# Autodesk Inventor assembly: !drivebay
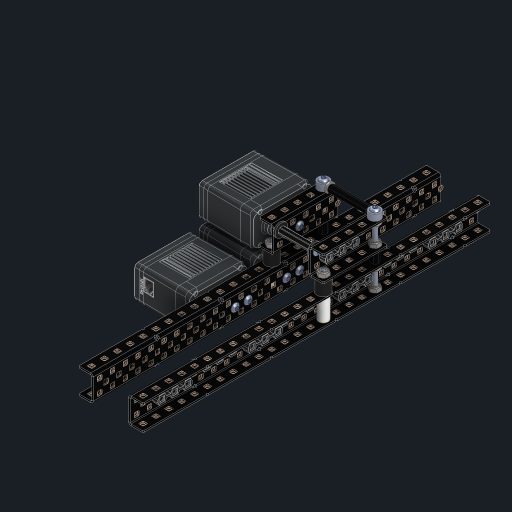
[picture p0: Inventor's stored thumbnail of the model, 512x512]
Saved by Autodesk Inventor 2024 (Build 280153000, 153)
## iProperties
Created: 2024-03-11
Part Number: !drivebay
Document SubType Name: Assembly
Designer: Averey Ku
Author: Averey Ku
## Documents named in this file (10)
- D:\vex_robotics\hardware\cad\eca\chassis\drivebay\!drivebay.iam
- D:\vex_robotics\hardware\cad\eca\chassis\drivebay\inner.iam
- D:\vex_robotics\hardware\cad\eca\chassis\drivebay\outer.iam
- D:\vex_robotics\hardware\cad\VEX-CAD-Inventor-1.41\Motion\Shaft LS\Shaft Collar ipts\Shaft Collar No Screw.ipt
- D:\vex_robotics\hardware\cad\VEX-CAD-Inventor-1.41\Structure\Standoff\Standoff 1.25.ipt
- D:\vex_robotics\hardware\cad\VEX-CAD-Inventor-1.41\Structure\Standoff\Standoff 1.50.ipt
- D:\vex_robotics\hardware\cad\VEX-CAD-Inventor-1.41\Structure\Standoff.ipt
- D:\vex_robotics\hardware\cad\VEX-CAD-Inventor-1.41\Motion\Spacers\Washer Delrin\DWasher .500 OD x .062500.ipt
- D:\vex_robotics\hardware\cad\VEX-CAD-Inventor-1.41\Motion\Spacers\Washer Steel\SWasher .375 OD x .062500.ipt
- D:\vex_robotics\hardware\cad\VEX-CAD-Inventor-1.41\Motion\Spacers\Washer Steel.ipt
## Components (9 placed, 7 different names)
1. inner:1 [sub-assembly] — Insert:1, Mate:1, Insert:2, Insert:8
2. outer:1 [sub-assembly] — Insert:1, Mate:1, Insert:3
3. Shaft Collar No Screw:1 — Insert:3, Mate:2
4. Shaft Collar No Screw:2 — Insert:2, Mate:2, Insert:5
5. Standoff 1.25:1 — Insert:6, Insert:7
6. Standoff 1.50:1 — Insert:4
7. DWasher .500 OD x .062500:1 — Insert:6
8. DWasher .500 OD x .062500:2 — Insert:7, Insert:8
9. SWasher .375 OD x .062500:1 — Insert:4, Insert:5
## Relationships (10: Insert 8, Mate 2)
- Insert:1 (34.925 mm): inner:1 ↔ outer:1
- Mate:1: inner:1 ↔ outer:1
- Insert:2: inner:1 ↔ Shaft Collar No Screw:2
- Insert:3: outer:1 ↔ Shaft Collar No Screw:1
- Mate:2: Shaft Collar No Screw:1 ↔ Shaft Collar No Screw:2
- Insert:4: Standoff 1.50:1 ↔ SWasher .375 OD x .062500:1
- Insert:5: Shaft Collar No Screw:2 ↔ SWasher .375 OD x .062500:1
- Insert:6: Standoff 1.25:1 ↔ DWasher .500 OD x .062500:1
- Insert:7: Standoff 1.25:1 ↔ DWasher .500 OD x .062500:2
- Insert:8: inner:1 ↔ DWasher .500 OD x .062500:2
